# Autodesk Inventor assembly: Accouplement moteur
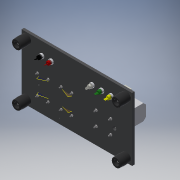
[picture p0: Inventor's stored thumbnail of the model, 180x180]
Saved by Autodesk Inventor 2016 SP1 (Build 200210100, 210)
## iProperties
Created: 2018-06-12
Part Number: Accouplement moteur
Material: Générique
Document SubType Name: Assembly
Designer: dimercur
Author: dimercur
## Documents named in this file (19)
- D:\Users\dimercur\Documents\git\dev-gei\dev-gei2\Accouplement Moteur 2015\Accouplement moteur.iam
- D:\Users\dimercur\Documents\git\dev-gei\dev-gei2\Accouplement Moteur 2015\Base2.ipt
- D:\Users\dimercur\Documents\git\dev-gei\dev-gei2\Accouplement Moteur 2015\Jambe_Crouzet.ipt
- D:\Users\dimercur\Documents\git\dev-gei\dev-gei2\Accouplement Moteur 2015\Moteur Crouzet.ipt
- D:\Users\dimercur\Documents\git\dev-gei\dev-gei2\Accouplement Moteur 2015\Ruland_PCMR25-9-8-A.iam
- D:\Users\dimercur\Documents\git\dev-gei\dev-gei2\Accouplement Moteur 2015\N2-0028-30-24.ipt
- D:\Users\dimercur\Documents\git\dev-gei\dev-gei2\Accouplement Moteur 2015\Jambe N2-0028.ipt
- D:\Users\dimercur\Documents\Inventor\Content Center Files\R2016\fr-FR\ISO 4762(2)\ISO 4762 - M5 x 16ISO.ipt
- D:\Users\dimercur\Documents\Inventor\Content Center Files\R2016\fr-FR\DIN EN ISO 4032\DIN EN ISO 4032 - M5.ipt
- D:\Users\dimercur\Documents\Inventor\Content Center Files\R2016\fr-FR\ISO 4762(2)\ISO 4762 - M4 x 12ISO.ipt
- D:\Users\dimercur\Documents\Inventor\Content Center Files\R2016\fr-FR\ISO 4762(2)\ISO 4762 - M3 x 20ISO.ipt
- D:\Users\dimercur\Documents\Inventor\Content Center Files\R2016\fr-FR\DIN EN ISO 4032\DIN EN ISO 4032 - M3,5.ipt
- D:\Users\dimercur\Documents\Inventor\Content Center Files\R2016\fr-FR\ISO 4762(2)\ISO 4762 - M4 x 20ISO.ipt
- D:\Users\dimercur\Documents\Inventor\Content Center Files\R2016\fr-FR\DIN EN ISO 4032\DIN EN ISO 4032 - M4.ipt
- D:\Users\dimercur\Documents\git\dev-gei\dev-gei2\Accouplement Moteur 2015\Prise banane.ipt
- D:\Users\dimercur\Documents\git\dev-gei\dev-gei2\Accouplement Moteur 2015\Pied.ipt
- D:\Users\dimercur\Documents\Inventor\Content Center Files\R2016\fr-FR\NF E 25-111\NF E 25-111 - M3.5x35 Classe de qualité 4.8.ipt
- D:\Users\dimercur\Documents\Inventor\Content Center Files\R2016\fr-FR\NF E 25-111\NF E 25-111 - M4x35 Classe de qualité 4.8.ipt
- D:\Users\dimercur\Documents\git\dev-gei\dev-gei2\Accouplement Moteur 2015\Bague Prise Banane.ipt
## Components (69 placed, 18 different names)
1. Base2:1 — Placage:1, Placage:3, Placage:4, Angle:1, Placage:12, Logement:25, Logement:26, Logement:27, Logement:28, Logement:29, Logement:30, Logement:31, Logement:32, Placage:15, Logement:37, Logement:38, Logement:39, Logement:40, Placage:17, Placage:18, Placage:19, Placage:20, Placage:21, Placage:22, Placage:23, Placage:24, Placage:25, Placage:26, Placage:27, Placage:28, Placage:29, Placage:30, Placage:31, Placage:32, Placage:33, Placage:34, Logement:41, Logement:42, Logement:43, Logement:44, Placage:41, Placage:42, Placage:43, Placage:44, Placage:45
2. Jambe_Crouzet:1 — Placage:1, Placage:3, Placage:4, Placage:5, Placage:6, Placage:7, Logement:13, Logement:14, Logement:15, Logement:16, Logement:17, Logement:18, Logement:19, Logement:20
3. Jambe_Crouzet:2 — Placage:8, Placage:9, Logement:9, Logement:10, Logement:11, Logement:12, Logement:21, Logement:22, Logement:23, Logement:24, Placage:16
4. Moteur Crouzet:1 — Placage:5, Placage:6, Placage:7, Placage:8, Placage:9, Placage:11, Placage:16
5. Ruland_PCMR25-9-8-A:1 [sub-assembly] — Placage:10, Placage:11
6. N2-0028-30-24:1 — Placage:10, Angle:1, Placage:13, Placage:14, Logement:1, Logement:2, Logement:3, Logement:4
7. Jambe N2-0028:1 — Placage:12, Placage:13, Placage:14, Logement:5, Logement:6, Logement:7, Logement:8, Placage:15, Logement:33, Logement:34, Logement:35, Logement:36
8. ISO 4762 M5 x 16:1 — Logement:1
9. ISO 4762 M5 x 16:2 — Logement:2
10. ISO 4762 M5 x 16:3 — Logement:3
11. ISO 4762 M5 x 16:4 — Logement:4
12. DIN EN ISO 4032 M5:1 — Logement:5
13. DIN EN ISO 4032 M5:2 — Logement:6
14. DIN EN ISO 4032 M5:3 — Logement:7
15. DIN EN ISO 4032 M5:4 — Logement:8
16. ISO 4762 M4 x 12:1 — Logement:9
17. ISO 4762 M4 x 12:2 — Logement:10
18. ISO 4762 M4 x 12:3 — Logement:11
19. ISO 4762 M4 x 12:4 — Logement:12
20. ISO 4762 M4 x 12:5 — Logement:13
21. ISO 4762 M4 x 12:6 — Logement:14
22. ISO 4762 M4 x 12:7 — Logement:15
23. ISO 4762 M4 x 12:8 — Logement:16
24. ISO 4762 M3 x 20:1 — Logement:17
25. ISO 4762 M3 x 20:2 — Logement:18
26. ISO 4762 M3 x 20:3 — Logement:19
27. ISO 4762 M3 x 20:4 — Logement:20
28. ISO 4762 M3 x 20:5 — Logement:21
29. ISO 4762 M3 x 20:6 — Logement:22
30. ISO 4762 M3 x 20:7 — Logement:23
31. ISO 4762 M3 x 20:8 — Logement:24
32. DIN EN ISO 4032 M3,5:1 — Logement:25
33. DIN EN ISO 4032 M3,5:2 — Logement:26
34. DIN EN ISO 4032 M3,5:3 — Logement:27
35. DIN EN ISO 4032 M3,5:4 — Logement:28
36. DIN EN ISO 4032 M3,5:5 — Logement:29
37. DIN EN ISO 4032 M3,5:6 — Logement:30
38. DIN EN ISO 4032 M3,5:7 — Logement:31
39. DIN EN ISO 4032 M3,5:8 — Logement:32
40. ISO 4762 M4 x 20:1 — Logement:33
41. ISO 4762 M4 x 20:2 — Logement:34
42. ISO 4762 M4 x 20:3 — Logement:35
43. ISO 4762 M4 x 20:4 — Logement:36
44. DIN EN ISO 4032 M4:1 — Logement:37
45. DIN EN ISO 4032 M4:2 — Logement:38
46. DIN EN ISO 4032 M4:3 — Logement:39
47. DIN EN ISO 4032 M4:4 — Logement:40
48. Prise banane:1 — Placage:17, Placage:22, Placage:40
49. Prise banane:2 — Placage:18, Placage:23, Placage:36
50. Prise banane:3 — Placage:19, Placage:24, Placage:37
51. Prise banane:4 — Placage:20, Placage:25, Placage:38
52. Prise banane:5 — Placage:21, Placage:26, Placage:39
53. Pied:1 — Placage:27, Placage:32, Logement:47
54. Pied:2 — Placage:28, Placage:31, Logement:46
55. Pied:3 — Placage:29, Placage:34, Logement:48
56. Pied:4 — Placage:30, Placage:33, Logement:45
57. NF E 25-111 M3.5x35 Classe de qualité 4.8:1 — Logement:41
58. NF E 25-111 M4x35 Classe de qualité 4.8:1 — Logement:42
59. NF E 25-111 M3.5x35 Classe de qualité 4.8:2 — Logement:43
60. NF E 25-111 M3.5x35 Classe de qualité 4.8:3 — Logement:44
61. DIN EN ISO 4032 M3,5:9 — Logement:45
62. DIN EN ISO 4032 M3,5:10 — Logement:46
63. DIN EN ISO 4032 M3,5:11 — Logement:47
64. DIN EN ISO 4032 M3,5:12 — Logement:48
65. Bague Prise Banane:1 — Placage:40, Placage:41
66. Bague Prise Banane:2 — Placage:36, Placage:42
67. Bague Prise Banane:3 — Placage:38, Placage:44
68. Bague Prise Banane:4 — Placage:37, Placage:43
69. Bague Prise Banane:5 — Placage:39, Placage:45
## Relationships (92: Insert 48, Mate 43, Angle 1)
- Placage:1 [Mate]: Base2:1 ↔ Jambe_Crouzet:1
- Placage:3 [Mate]: Base2:1 ↔ Jambe_Crouzet:1
- Placage:4 [Mate]: Base2:1 ↔ Jambe_Crouzet:1
- Placage:5 [Mate]: Jambe_Crouzet:1 ↔ Moteur Crouzet:1
- Placage:6 [Mate]: Jambe_Crouzet:1 ↔ Moteur Crouzet:1
- Placage:7 [Mate]: Jambe_Crouzet:1 ↔ Moteur Crouzet:1
- Placage:8 [Mate]: Jambe_Crouzet:2 ↔ Moteur Crouzet:1
- Placage:9 [Mate]: Jambe_Crouzet:2 ↔ Moteur Crouzet:1
- Placage:10 [Mate]: Ruland_PCMR25-9-8-A:1 ↔ N2-0028-30-24:1
- Placage:11 [Mate]: Moteur Crouzet:1 ↔ Ruland_PCMR25-9-8-A:1
- Angle:1 (0 deg): Base2:1 ↔ N2-0028-30-24:1
- Placage:12 [Mate]: Base2:1 ↔ Jambe N2-0028:1
- Placage:13 [Mate]: N2-0028-30-24:1 ↔ Jambe N2-0028:1
- Placage:14 [Mate]: N2-0028-30-24:1 ↔ Jambe N2-0028:1
- Logement:1 [Insert]: N2-0028-30-24:1 ↔ ISO 4762 M5 x 16:1
- Logement:2 [Insert]: N2-0028-30-24:1 ↔ ISO 4762 M5 x 16:2
- Logement:3 [Insert]: N2-0028-30-24:1 ↔ ISO 4762 M5 x 16:3
- Logement:4 [Insert]: N2-0028-30-24:1 ↔ ISO 4762 M5 x 16:4
- Logement:5 [Insert]: Jambe N2-0028:1 ↔ DIN EN ISO 4032 M5:1
- Logement:6 [Insert]: Jambe N2-0028:1 ↔ DIN EN ISO 4032 M5:2
- Logement:7 [Insert]: Jambe N2-0028:1 ↔ DIN EN ISO 4032 M5:3
- Logement:8 [Insert]: Jambe N2-0028:1 ↔ DIN EN ISO 4032 M5:4
- Logement:9 [Insert]: Jambe_Crouzet:2 ↔ ISO 4762 M4 x 12:1
- Logement:10 [Insert]: Jambe_Crouzet:2 ↔ ISO 4762 M4 x 12:2
- Logement:11 [Insert]: Jambe_Crouzet:2 ↔ ISO 4762 M4 x 12:3
- Logement:12 [Insert]: Jambe_Crouzet:2 ↔ ISO 4762 M4 x 12:4
- Logement:13 [Insert]: Jambe_Crouzet:1 ↔ ISO 4762 M4 x 12:5
- Logement:14 [Insert]: Jambe_Crouzet:1 ↔ ISO 4762 M4 x 12:6
- Logement:15 [Insert]: Jambe_Crouzet:1 ↔ ISO 4762 M4 x 12:7
- Logement:16 [Insert]: Jambe_Crouzet:1 ↔ ISO 4762 M4 x 12:8
- Logement:17 [Insert]: Jambe_Crouzet:1 ↔ ISO 4762 M3 x 20:1
- Logement:18 [Insert]: Jambe_Crouzet:1 ↔ ISO 4762 M3 x 20:2
- Logement:19 [Insert]: Jambe_Crouzet:1 ↔ ISO 4762 M3 x 20:3
- Logement:20 [Insert]: Jambe_Crouzet:1 ↔ ISO 4762 M3 x 20:4
- Logement:21 [Insert]: Jambe_Crouzet:2 ↔ ISO 4762 M3 x 20:5
- Logement:22 [Insert]: Jambe_Crouzet:2 ↔ ISO 4762 M3 x 20:6
- Logement:23 [Insert]: Jambe_Crouzet:2 ↔ ISO 4762 M3 x 20:7
- Logement:24 [Insert]: Jambe_Crouzet:2 ↔ ISO 4762 M3 x 20:8
- Logement:25 [Insert]: Base2:1 ↔ DIN EN ISO 4032 M3,5:1
- Logement:26 [Insert]: Base2:1 ↔ DIN EN ISO 4032 M3,5:2
- Logement:27 [Insert]: Base2:1 ↔ DIN EN ISO 4032 M3,5:3
- Logement:28 [Insert]: Base2:1 ↔ DIN EN ISO 4032 M3,5:4
- Logement:29 [Insert]: Base2:1 ↔ DIN EN ISO 4032 M3,5:5
- Logement:30 [Insert]: Base2:1 ↔ DIN EN ISO 4032 M3,5:6
- Logement:31 [Insert]: Base2:1 ↔ DIN EN ISO 4032 M3,5:7
- Logement:32 [Insert]: Base2:1 ↔ DIN EN ISO 4032 M3,5:8
- Placage:15 [Mate]: Base2:1 ↔ Jambe N2-0028:1
- Logement:33 [Insert]: Jambe N2-0028:1 ↔ ISO 4762 M4 x 20:1
- Logement:34 [Insert]: Jambe N2-0028:1 ↔ ISO 4762 M4 x 20:2
- Logement:35 [Insert]: Jambe N2-0028:1 ↔ ISO 4762 M4 x 20:3
- Logement:36 [Insert]: Jambe N2-0028:1 ↔ ISO 4762 M4 x 20:4
- Logement:37 [Insert]: Base2:1 ↔ DIN EN ISO 4032 M4:1
- Logement:38 [Insert]: Base2:1 ↔ DIN EN ISO 4032 M4:2
- Logement:39 [Insert]: Base2:1 ↔ DIN EN ISO 4032 M4:3
- Logement:40 [Insert]: Base2:1 ↔ DIN EN ISO 4032 M4:4
- Placage:16 [Mate]: Jambe_Crouzet:2 ↔ Moteur Crouzet:1
- Placage:17 [Mate]: Base2:1 ↔ Prise banane:1
- Placage:18 [Mate]: Base2:1 ↔ Prise banane:2
- Placage:19 [Mate]: Base2:1 ↔ Prise banane:3
- Placage:20 [Mate]: Base2:1 ↔ Prise banane:4
- Placage:21 [Mate]: Base2:1 ↔ Prise banane:5
- Placage:22 [Mate]: Base2:1 ↔ Prise banane:1
- Placage:23 [Mate]: Base2:1 ↔ Prise banane:2
- Placage:24 [Mate]: Base2:1 ↔ Prise banane:3
- Placage:25 [Mate]: Base2:1 ↔ Prise banane:4
- Placage:26 [Mate]: Base2:1 ↔ Prise banane:5
- Placage:27 [Mate]: Base2:1 ↔ Pied:1
- Placage:28 [Mate]: Base2:1 ↔ Pied:2
- Placage:29 [Mate]: Base2:1 ↔ Pied:3
- Placage:30 [Mate]: Base2:1 ↔ Pied:4
- Placage:31 [Mate]: Base2:1 ↔ Pied:2
- Placage:32 [Mate]: Base2:1 ↔ Pied:1
- Placage:33 [Mate]: Base2:1 ↔ Pied:4
- Placage:34 [Mate]: Base2:1 ↔ Pied:3
- Logement:41 [Insert]: Base2:1 ↔ NF E 25-111 M3.5x35 Classe de qualité 4.8:1
- Logement:42 [Insert]: Base2:1 ↔ NF E 25-111 M4x35 Classe de qualité 4.8:1
- Logement:43 [Insert]: Base2:1 ↔ NF E 25-111 M3.5x35 Classe de qualité 4.8:2
- Logement:44 [Insert]: Base2:1 ↔ NF E 25-111 M3.5x35 Classe de qualité 4.8:3
- Logement:45 [Insert]: Pied:4 ↔ DIN EN ISO 4032 M3,5:9
- Logement:46 [Insert]: Pied:2 ↔ DIN EN ISO 4032 M3,5:10
- Logement:47 [Insert]: Pied:1 ↔ DIN EN ISO 4032 M3,5:11
- Logement:48 [Insert]: Pied:3 ↔ DIN EN ISO 4032 M3,5:12
- Placage:36 [Mate]: Prise banane:2 ↔ Bague Prise Banane:2
- Placage:37 [Mate]: Prise banane:3 ↔ Bague Prise Banane:4
- Placage:38 [Mate]: Prise banane:4 ↔ Bague Prise Banane:3
- Placage:39 [Mate]: Prise banane:5 ↔ Bague Prise Banane:5
- Placage:40 [Mate]: Prise banane:1 ↔ Bague Prise Banane:1
- Placage:41 [Mate]: Base2:1 ↔ Bague Prise Banane:1
- Placage:42 [Mate]: Base2:1 ↔ Bague Prise Banane:2
- Placage:43 [Mate]: Base2:1 ↔ Bague Prise Banane:4
- Placage:44 [Mate]: Base2:1 ↔ Bague Prise Banane:3
- Placage:45 [Mate]: Base2:1 ↔ Bague Prise Banane:5
